# Autodesk Inventor assembly: SKF_NKX 10 ZTN
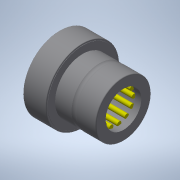
[picture p0: Inventor's stored thumbnail of the model, 180x180]
Saved by Autodesk Inventor 2022 (Build 260153000, 153)
## iProperties
Category: PARTsolutions
Company: SKF
Created: 2022-07-21
Part Number: SKF_NKX 10 ZTN
Catalog Web Link: www.cadenas.de
Description: BVN_002_003-Needle roller / thrust rolling bearings
Vendor: SKF
Document SubType Name: Assembly
Designer: psAdmin
Manufacturer: SKF
Mass: 36 g
Surface Area: 59.471 cm^2
Volume: 5.6714 cm^3
Density: 6.34764 g/cm^3
PSOL_IDENT_0: {$CADENAS_DATA/23d-libs/skf/bearings_units_and_housings/roller_bearings/needle_roller_bearings/bvn_0
PSOL_IDENT_1: 02_003.prj},176 {VTYP=3D},{NB=SKF_NKX 10 ZTN},{LINA=SKF_NKX 10 ZTN},{NN=BVN_002_003},{DATE=08.07.202
PSOL_IDENT_2: 2 10:25:50},{GEOMDATE=06.12.2021 10:15:46},{VERSION=},{LINEID=10190},{WBVAR=},{WBNUMERIC=}  {NB=SKF_
PSOL_IDENT_3: NKX 10 ZTN},{LINA=SKF_NKX 10 ZTN},{KT=DUMMY},{DESIGNATION=NKX 10 ZTN},{DESIGN=comb_nkxz},{SB=ball},{
PSOL_IDENT_4: DESIGNZ=1},{F=10},{FW=10},{FALG=10.000},{D=19.000},{C=23.000},{C1=9},{C2=6.5},{DD=10.000},{D1=24.1},
PSOL_IDENT_5: {D2=25.200},{R12=0.300},{PITCH=11.500},{PITCHA=11.500},{ALPHAA=0.000},{DW=1.500},{DWA=4.762},{LW=10.
PSOL_IDENT_6: 800},{LWA=0.000},{DA=19.700},{LOAD1=5.940},{LOAD2=8.000},{LOAD3=9.950},{LOAD4=15.300},{LOAD5=0.900},
PSOL_IDENT_7: {LOAD6=0.560},{LOADA=0.0},{SPEED1=9500},{SPEED2=8000},{Z=13.000},{ZA=13.000},{II=1.000},{IIA=1.000},
PSOL_IDENT_8: {MASS=0.036},{C3=0.000},{C1A=9},{DAMAX=},{SPEED1X=28000},{RAMAX=0.3},{IIX=1},{LWX=},{LOAD4X=},{SPEED
PSOL_IDENT_9: 2X=32000},{ZX=10},{LOAD6X=},{ALPHAX=},{LOAD3X=},{ALPHA=90},{RBMAX=0.3},{DWXX=},{PITCHXX=11.5},{DI=7}
PSOL_IDENT_10: ,{DDAMIN=19.7},{DWX=4.762},{C1X=6.5},{ZXX=13},{LOADAX=},{POPULAR=},{PITCHX=17},{BI=16},{D1ALG=24.100
PSOL_IDENT_11: },{C2ALG=6.500},{PITCHXXA=11.500},{LWXA=0.000},{DWXXA=0.000},{DIA=7.000}
NB: SKF_NKX 10 ZTN
NN: BVN_002_003
NT: Needle roller / thrust rolling bearings
NBSYN: SKF_$DESIGNATION.
LINA: SKF_NKX 10 ZTN
CATALOG: SKF
DESIGNATION: NKX 10 ZTN
F: 10
D: 19
C: 23
C1: 9
C2: 6.5
DD: 10
D2: 25.2
R12: 0.3
LOAD1: 5.94
LOAD2: 8
LOAD3: 9.95
LOAD4: 15.3
LOAD5: 0.9
LOAD6: 0.56
LOADA: 0
SPEED1: 9500
SPEED2: 8000
MASS: 0.036
SUPPLIER: SKF
ARTICLENO: SKF_NKX 10 ZTN
BOMINFO: SKF_NKX 10 ZTN
CREATOR: CADENAS GmbH
NKX_10_RadialPart_Width: 14,000 mm
NKX_10_AxialPart_Width: 9,000 mm
NKX_10_MaxOuterDia: 25,200 mm
NKX_10_RiadialPart_Dia: 19,000 mm
Title: SKF_NKX 10 ZTN
Author: Cadenas PARTsolutions
Comments: Needle roller / thrust rolling bearings
## Documents named in this file (4)
- C:\Users\alexw\Documents\Inventor\Projects\03_CurrentProjects\MasterThesis\Parallelsystem_DaVinci_CAD\Downloads\SKF_NKX 10 ZTN\SKF_NKX 10 ZTN.iam
- C:\Users\alexw\Documents\Inventor\Projects\03_CurrentProjects\MasterThesis\Parallelsystem_DaVinci_CAD\Downloads\SKF_NKX 10 ZTN\SKF_NKX 10 ZTN_PART1.ipt
- C:\Users\alexw\Documents\Inventor\Projects\03_CurrentProjects\MasterThesis\Parallelsystem_DaVinci_CAD\Downloads\SKF_NKX 10 ZTN\SKF_NKX 10 ZTN_PART2.ipt
- C:\Users\alexw\Documents\Inventor\Projects\03_CurrentProjects\MasterThesis\Parallelsystem_DaVinci_CAD\Downloads\SKF_NKX 10 ZTN\SKF_NKX 10 ZTN_PART3.ipt
## Components (27 placed, 3 different names)
1. SKF_NKX 10 ZTN_PART1:1
2. SKF_NKX 10 ZTN_PART2:1
3. SKF_NKX 10 ZTN_PART2:2
4. SKF_NKX 10 ZTN_PART2:3
5. SKF_NKX 10 ZTN_PART2:4
6. SKF_NKX 10 ZTN_PART2:5
7. SKF_NKX 10 ZTN_PART2:6
8. SKF_NKX 10 ZTN_PART2:7
9. SKF_NKX 10 ZTN_PART2:8
10. SKF_NKX 10 ZTN_PART2:9
11. SKF_NKX 10 ZTN_PART2:10
12. SKF_NKX 10 ZTN_PART2:11
13. SKF_NKX 10 ZTN_PART2:12
14. SKF_NKX 10 ZTN_PART2:13
15. SKF_NKX 10 ZTN_PART3:1
16. SKF_NKX 10 ZTN_PART3:2
17. SKF_NKX 10 ZTN_PART3:3
18. SKF_NKX 10 ZTN_PART3:4
19. SKF_NKX 10 ZTN_PART3:5
20. SKF_NKX 10 ZTN_PART3:6
21. SKF_NKX 10 ZTN_PART3:7
22. SKF_NKX 10 ZTN_PART3:8
23. SKF_NKX 10 ZTN_PART3:9
24. SKF_NKX 10 ZTN_PART3:10
25. SKF_NKX 10 ZTN_PART3:11
26. SKF_NKX 10 ZTN_PART3:12
27. SKF_NKX 10 ZTN_PART3:13
## Named parameters: NKX_10_RadialPart_Width = 14 mm, NKX_10_AxialPart_Width = 9 mm, NKX_10_MaxOuterDia = 25.2 mm, NKX_10_RiadialPart_Dia = 19 mm
